# Autodesk Inventor assembly: 000.300 - Опора поворотная
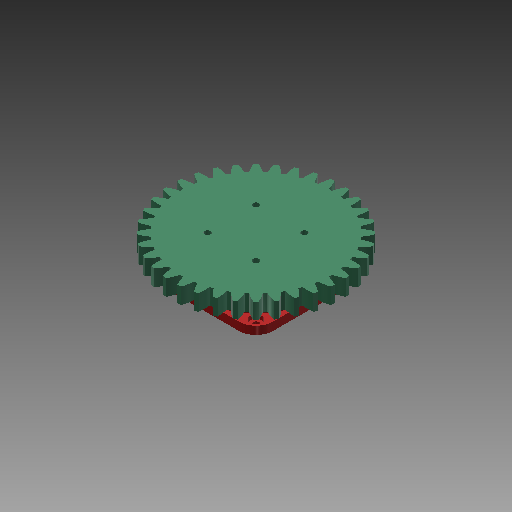
[picture p0: Inventor's stored thumbnail of the model, 512x512]
Saved by Autodesk Inventor 2019 (Build 230136000, 136)
## iProperties
Created: 2020-02-27
Part Number: 000.300 - Опора поворотная
Material: Типовые
Document SubType Name: Assembly
Designer: Петров Иван
Author: Петров Иван
## Documents named in this file (4)
- E:\IVAN\Ivan_desktop\GitHub\Manipulation_IRS\hardware\5-DOF\000.300 - Опора поворотная.iam
- E:\IVAN\Ivan_desktop\GitHub\Manipulation_IRS\hardware\5-DOF\000.301 - База подшипника.ipt
- E:\IVAN\Ivan_desktop\GitHub\Manipulation_IRS\hardware\5-DOF\components\Подшипник 25х47х8 7000105.ipt
- E:\IVAN\Ivan_desktop\GitHub\Manipulation_IRS\hardware\5-DOF\000.302 - Втулка.ipt
## Components (3 placed, 3 different names)
1. 000.301 - База подшипника:1 — Совмещение:1, Совмещение:2
2. Подшипник 25х47х8 7000105:1 — Совмещение:1, Совмещение:2, Совмещение:3, Совмещение:4
3. 000.302 - Втулка:1 — Совмещение:3, Совмещение:4
## Relationships (4: Mate 4)
- Совмещение:1 [Mate]: 000.301 - База подшипника:1 ↔ Подшипник 25х47х8 7000105:1
- Совмещение:2 [Mate]: 000.301 - База подшипника:1 ↔ Подшипник 25х47х8 7000105:1
- Совмещение:3 [Mate]: Подшипник 25х47х8 7000105:1 ↔ 000.302 - Втулка:1
- Совмещение:4 [Mate]: Подшипник 25х47х8 7000105:1 ↔ 000.302 - Втулка:1
